# Autodesk Inventor assembly: Connectique
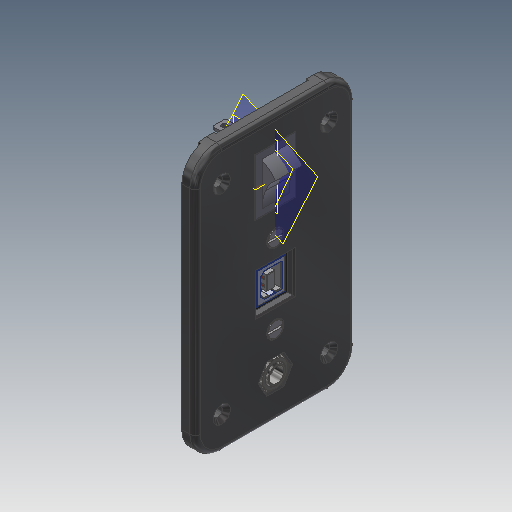
[picture p0: Inventor's stored thumbnail of the model, 512x512]
Saved by Autodesk Inventor 2017 (Build 210142000, 142)
## iProperties
Company: FABLAB Frenchmakers
Part Number: Connectique
Material: Générique
Document SubType Name: Assembly
Designer: FABLAB Frenchmakers
Project: 1420 Vauban 3D XL
Catalog Web Link: http://frenchmakers.com/
Stock Number: 1420-09-00
## Documents named in this file (7)
- W:\Professionnel\Conception FABLAB\1420-Vauban 3D XL\1420-09 Connectique\1420-09-00 Connectique.iam
- W:\Professionnel\Conception FABLAB\1420-Vauban 3D XL\1420-09 Connectique\1420-09-04 Support connectique.ipt
- W:\Professionnel\Conception FABLAB\1420-Vauban 3D XL\1420-09 Connectique\1420-09-01 Plug alimentation.ipt
- W:\Professionnel\Conception FABLAB\1420-Vauban 3D XL\1420-09 Connectique\1420-09-03 Ecrou plug alimentation.ipt
- W:\Professionnel\Conception FABLAB\1420-Vauban 3D XL\1420-09 Connectique\1420-09-10 Bouton\1420-09-03 Bouton.iam
- W:\Professionnel\Conception FABLAB\1420-Vauban 3D XL\1420-09 Connectique\1420-09-02 Prise USB.ipt
- W:\Professionnel\Conception FABLAB\1420-Vauban 3D XL\1420-90 Centre de contenu\fr-FR\DIN 963\DIN 963 - M3 x 8.ipt
## Components (7 placed, 6 different names)
1. 1420-09-04 Support connectique:1 — Logement:1, Logement:2, Angle:1, Placage:1, Placage:2, Placage:3, Logement:3, Logement:4, Logement:5, Logement:6
2. 1420-09-01 Plug alimentation:1 — Logement:1
3. 1420-09-03 Ecrou plug alimentation:1 — Logement:2, Angle:1
4. 1420-09-03 Bouton:1 [sub-assembly] — Placage:1, Placage:2, Placage:3
5. 1420-09-02 Prise USB:1 — Logement:3, Logement:4
6. DIN 963 - Remplacé par DIN EN ISO 2009 M3 x 8:2 — Logement:6
7. DIN 963 - Remplacé par DIN EN ISO 2009 M3 x 8:1 — Logement:5
## Relationships (10: Insert 6, Mate 3, Angle 1)
- Logement:1 [Insert]: 1420-09-04 Support connectique:1 ↔ 1420-09-01 Plug alimentation:1
- Logement:2 [Insert]: 1420-09-04 Support connectique:1 ↔ 1420-09-03 Ecrou plug alimentation:1
- Angle:1 (0 deg): 1420-09-04 Support connectique:1 ↔ 1420-09-03 Ecrou plug alimentation:1
- Placage:1 [Mate]: 1420-09-04 Support connectique:1 ↔ 1420-09-03 Bouton:1
- Placage:2 [Mate] (0.25 mm): 1420-09-04 Support connectique:1 ↔ 1420-09-03 Bouton:1
- Placage:3 [Mate] (0.25 mm): 1420-09-04 Support connectique:1 ↔ 1420-09-03 Bouton:1
- Logement:3 [Insert]: 1420-09-04 Support connectique:1 ↔ 1420-09-02 Prise USB:1
- Logement:4 [Insert]: 1420-09-04 Support connectique:1 ↔ 1420-09-02 Prise USB:1
- Logement:5 [Insert]: 1420-09-04 Support connectique:1 ↔ DIN 963 - Remplacé par DIN EN ISO 2009 M3 x 8:1
- Logement:6 [Insert]: 1420-09-04 Support connectique:1 ↔ DIN 963 - Remplacé par DIN EN ISO 2009 M3 x 8:2
